# Autodesk Inventor assembly: A2017_T5_09
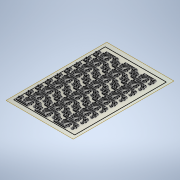
[picture p0: Inventor's stored thumbnail of the model, 180x180]
Saved by Autodesk Inventor 2022.3 (Build 263350000, 350)
## iProperties
Created: 2022-09-28
Part Number: A2017_T5_09
Document SubType Name: Assembly
Designer: Masato
Author: Masato
## Documents named in this file (3)
- C:\Users\Masato\Documents\Inventor\Inventor for CIT Brains\SUSTAINA-OP - cam\Cam\A2017_T5\A2017_T5_09.iam
- C:\Users\Masato\Documents\Inventor\Inventor for CIT Brains\SUSTAINA-OP - cam\Cam\DisposableBoard.ipt
- C:\Users\Masato\Documents\Inventor\Inventor for CIT Brains\SUSTAINA-OP - cam\LowerBody\Ankle\Ankle_back_frame.ipt
## Components (55 placed, 2 different names)
1. DisposableBoard:1 — フラッシュ:1, フラッシュ:2, フラッシュ:3, フラッシュ:4, フラッシュ:5, フラッシュ:6
2. Ankle_back_frame:1 — メイト:1, フラッシュ:5, フラッシュ:6, 正接:2, 角度:1, 正接:3
3. Ankle_back_frame:2 — メイト:2, 正接:2, 角度:1, 正接:3
4. Ankle_back_frame:3
5. Ankle_back_frame:4
6. Ankle_back_frame:5
7. Ankle_back_frame:6
8. Ankle_back_frame:7
9. Ankle_back_frame:8
10. Ankle_back_frame:9
11. Ankle_back_frame:10
12. Ankle_back_frame:11
13. Ankle_back_frame:12
14. Ankle_back_frame:13
15. Ankle_back_frame:14
16. Ankle_back_frame:15
17. Ankle_back_frame:16
18. Ankle_back_frame:17
19. Ankle_back_frame:18
20. Ankle_back_frame:19
21. Ankle_back_frame:20
22. Ankle_back_frame:21
23. Ankle_back_frame:22
24. Ankle_back_frame:23
25. Ankle_back_frame:24
26. Ankle_back_frame:25
27. Ankle_back_frame:26
28. Ankle_back_frame:27
29. Ankle_back_frame:28
30. Ankle_back_frame:29
31. Ankle_back_frame:30
32. Ankle_back_frame:31
33. Ankle_back_frame:32
34. Ankle_back_frame:33
35. Ankle_back_frame:34
36. Ankle_back_frame:35
37. Ankle_back_frame:36
38. Ankle_back_frame:37
39. Ankle_back_frame:38
40. Ankle_back_frame:39
41. Ankle_back_frame:40
42. Ankle_back_frame:41
43. Ankle_back_frame:42
44. Ankle_back_frame:43
45. Ankle_back_frame:44
46. Ankle_back_frame:45
47. Ankle_back_frame:46
48. Ankle_back_frame:47
49. Ankle_back_frame:48
50. Ankle_back_frame:49
51. Ankle_back_frame:50
52. Ankle_back_frame:51
53. Ankle_back_frame:52
54. Ankle_back_frame:53
55. Ankle_back_frame:54
## Component patterns: (27 elements, first: Ankle_back_frame:1 + Ankle_back_frame:2)
## Relationships (11: Flush 6, Mate 2, Tangent 2, Angle 1)
- フラッシュ:1 [Flush]: DisposableBoard:1
- フラッシュ:2 [Flush]: DisposableBoard:1
- フラッシュ:3 [Flush]: DisposableBoard:1
- フラッシュ:4 [Flush]: DisposableBoard:1
- メイト:1 [Mate]: Ankle_back_frame:1
- フラッシュ:5 [Flush] (2 mm): DisposableBoard:1 ↔ Ankle_back_frame:1
- フラッシュ:6 [Flush] (-2 mm): DisposableBoard:1 ↔ Ankle_back_frame:1
- メイト:2 [Mate]: Ankle_back_frame:2
- 正接:2 [Tangent] (2.1 mm): Ankle_back_frame:1 ↔ Ankle_back_frame:2
- 角度:1 [Angle] (0 deg): Ankle_back_frame:1 ↔ Ankle_back_frame:2
- 正接:3 [Tangent] (-2.1 mm): Ankle_back_frame:1 ↔ Ankle_back_frame:2
